# Autodesk Inventor assembly: Assembly1
(part 5 of 8)
- Mate:747: FRAME:1 ↔ disk holder:133
- Mate:748: FRAME:1 ↔ disk holder:134
- Mate:749: FRAME:1 ↔ disk holder:135
- Mate:750: FRAME:1 ↔ disk holder:136
- [RevoluteJoint]: disk holder:137 ↔ coin:137
- [Angle] (-25 deg): disk holder:137 ↔ coin:137
- [Mate]: disk holder:137 ↔ Coil:273
- [Mate]: disk holder:137 ↔ Coil:273
- [Angle] (270 deg): disk holder:137 ↔ Coil:273
- [Mate]: disk holder:137 ↔ Coil:274
- [Angle] (270 deg): disk holder:137 ↔ Coil:274
- [Mate]: disk holder:137 ↔ Coil:274
- [RevoluteJoint]: disk holder:138 ↔ coin:138
- [Angle] (-25 deg): disk holder:138 ↔ coin:138
- [Mate]: disk holder:138 ↔ Coil:275
- [Mate]: disk holder:138 ↔ Coil:275
- [Angle] (270 deg): disk holder:138 ↔ Coil:275
- [Mate]: disk holder:138 ↔ Coil:276
- [Angle] (270 deg): disk holder:138 ↔ Coil:276
- [Mate]: disk holder:138 ↔ Coil:276
- [RevoluteJoint]: disk holder:139 ↔ coin:139
- [Angle] (-25 deg): disk holder:139 ↔ coin:139
- [Mate]: disk holder:139 ↔ Coil:277
- [Mate]: disk holder:139 ↔ Coil:277
- [Angle] (270 deg): disk holder:139 ↔ Coil:277
- [Mate]: disk holder:139 ↔ Coil:278
- [Angle] (270 deg): disk holder:139 ↔ Coil:278
- [Mate]: disk holder:139 ↔ Coil:278
- [RevoluteJoint]: disk holder:140 ↔ coin:140
- [Angle] (-25 deg): disk holder:140 ↔ coin:140
- [Mate]: disk holder:140 ↔ Coil:279
- [Mate]: disk holder:140 ↔ Coil:279
- [Angle] (270 deg): disk holder:140 ↔ Coil:279
- [Mate]: disk holder:140 ↔ Coil:280
- [Angle] (270 deg): disk holder:140 ↔ Coil:280
- [Mate]: disk holder:140 ↔ Coil:280
- [RevoluteJoint]: disk holder:141 ↔ coin:141
- [Angle] (-25 deg): disk holder:141 ↔ coin:141
- [Mate]: disk holder:141 ↔ Coil:281
- [Mate]: disk holder:141 ↔ Coil:281
- [Angle] (270 deg): disk holder:141 ↔ Coil:281
- [Mate]: disk holder:141 ↔ Coil:282
- [Angle] (270 deg): disk holder:141 ↔ Coil:282
- [Mate]: disk holder:141 ↔ Coil:282
- [RevoluteJoint]: disk holder:142 ↔ coin:142
- [Angle] (-25 deg): disk holder:142 ↔ coin:142
- [Mate]: disk holder:142 ↔ Coil:283
- [Mate]: disk holder:142 ↔ Coil:283
- [Angle] (270 deg): disk holder:142 ↔ Coil:283
- [Mate]: disk holder:142 ↔ Coil:284
- [Angle] (270 deg): disk holder:142 ↔ Coil:284
- [Mate]: disk holder:142 ↔ Coil:284
- Flush:213: disk holder:137 ↔ disk holder:138
- Flush:214: disk holder:138 ↔ disk holder:139
- Flush:215: disk holder:139 ↔ disk holder:140
- Flush:216: disk holder:140 ↔ disk holder:141
- Flush:217: disk holder:141 ↔ disk holder:142
- Flush:218: FRAME:1 ↔ disk holder:137
- Flush:219: disk holder:137 ↔ disk holder:138
- Flush:220: disk holder:138 ↔ disk holder:139
- Flush:221: disk holder:139 ↔ disk holder:140
- Flush:222: disk holder:140 ↔ disk holder:141
- Flush:223: disk holder:141 ↔ disk holder:142
- Mate:775: FRAME:1 ↔ disk holder:137
- Mate:776: FRAME:1 ↔ disk holder:137
- Mate:777: FRAME:1 ↔ disk holder:138
- Mate:778: FRAME:1 ↔ disk holder:139
- Mate:779: FRAME:1 ↔ disk holder:140
- Mate:780: FRAME:1 ↔ disk holder:141
- Mate:781: FRAME:1 ↔ disk holder:142
- [RevoluteJoint]: disk holder:143 ↔ coin:143
- [Angle] (-25 deg): disk holder:143 ↔ coin:143
- [Mate]: disk holder:143 ↔ Coil:285
- [Mate]: disk holder:143 ↔ Coil:285
- [Angle] (270 deg): disk holder:143 ↔ Coil:285
- [Mate]: disk holder:143 ↔ Coil:286
- [Angle] (270 deg): disk holder:143 ↔ Coil:286
- [Mate]: disk holder:143 ↔ Coil:286
- [RevoluteJoint]: disk holder:144 ↔ coin:144
- [Angle] (-25 deg): disk holder:144 ↔ coin:144
- [Mate]: disk holder:144 ↔ Coil:287
- [Mate]: disk holder:144 ↔ Coil:287
- [Angle] (270 deg): disk holder:144 ↔ Coil:287
- [Mate]: disk holder:144 ↔ Coil:288
- [Angle] (270 deg): disk holder:144 ↔ Coil:288
- [Mate]: disk holder:144 ↔ Coil:288
- [RevoluteJoint]: disk holder:145 ↔ coin:145
- [Angle] (-25 deg): disk holder:145 ↔ coin:145
- [Mate]: disk holder:145 ↔ Coil:289
- [Mate]: disk holder:145 ↔ Coil:289
- [Angle] (270 deg): disk holder:145 ↔ Coil:289
- [Mate]: disk holder:145 ↔ Coil:290
- [Angle] (270 deg): disk holder:145 ↔ Coil:290
- [Mate]: disk holder:145 ↔ Coil:290
- [RevoluteJoint]: disk holder:146 ↔ coin:146
- [Angle] (-25 deg): disk holder:146 ↔ coin:146
- [Mate]: disk holder:146 ↔ Coil:291
- [Mate]: disk holder:146 ↔ Coil:291
- [Angle] (270 deg): disk holder:146 ↔ Coil:291
- [Mate]: disk holder:146 ↔ Coil:292
- [Angle] (270 deg): disk holder:146 ↔ Coil:292
- [Mate]: disk holder:146 ↔ Coil:292
- [RevoluteJoint]: disk holder:147 ↔ coin:147
- [Angle] (-25 deg): disk holder:147 ↔ coin:147
- [Mate]: disk holder:147 ↔ Coil:293
- [Mate]: disk holder:147 ↔ Coil:293
- [Angle] (270 deg): disk holder:147 ↔ Coil:293
- [Mate]: disk holder:147 ↔ Coil:294
- [Angle] (270 deg): disk holder:147 ↔ Coil:294
- [Mate]: disk holder:147 ↔ Coil:294
- [RevoluteJoint]: disk holder:148 ↔ coin:148
- [Angle] (-25 deg): disk holder:148 ↔ coin:148
- [Mate]: disk holder:148 ↔ Coil:295
- [Mate]: disk holder:148 ↔ Coil:295
- [Angle] (270 deg): disk holder:148 ↔ Coil:295
- [Mate]: disk holder:148 ↔ Coil:296
- [Angle] (270 deg): disk holder:148 ↔ Coil:296
- [Mate]: disk holder:148 ↔ Coil:296
- Flush:224: disk holder:143 ↔ disk holder:144
- Flush:225: disk holder:144 ↔ disk holder:145
- Flush:226: disk holder:145 ↔ disk holder:146
- Flush:227: disk holder:146 ↔ disk holder:147
- Flush:228: disk holder:147 ↔ disk holder:148
- Flush:229: FRAME:1 ↔ disk holder:143
- Mate:806: FRAME:1 ↔ disk holder:143
- Mate:807: disk holder:143 ↔ disk holder:144
- Mate:808: disk holder:144 ↔ disk holder:145
- Mate:809: disk holder:145 ↔ disk holder:146
- Mate:810: disk holder:146 ↔ disk holder:147
- Mate:811: disk holder:147 ↔ disk holder:148
- Mate:812: FRAME:1 ↔ disk holder:143
- Mate:813: FRAME:1 ↔ disk holder:144
- Mate:814: FRAME:1 ↔ disk holder:145
- Mate:815: FRAME:1 ↔ disk holder:146
- Mate:816: FRAME:1 ↔ disk holder:147
- Mate:817: FRAME:1 ↔ disk holder:148
- [RevoluteJoint]: disk holder:149 ↔ coin:149
- [Angle] (-25 deg): disk holder:149 ↔ coin:149
- [Mate]: disk holder:149 ↔ Coil:297
- [Mate]: disk holder:149 ↔ Coil:297
- [Angle] (270 deg): disk holder:149 ↔ Coil:297
- [Mate]: disk holder:149 ↔ Coil:298
- [Angle] (270 deg): disk holder:149 ↔ Coil:298
- [Mate]: disk holder:149 ↔ Coil:298
- [RevoluteJoint]: disk holder:150 ↔ coin:150
- [Angle] (-25 deg): disk holder:150 ↔ coin:150
- [Mate]: disk holder:150 ↔ Coil:299
- [Mate]: disk holder:150 ↔ Coil:299
- [Angle] (270 deg): disk holder:150 ↔ Coil:299
- [Mate]: disk holder:150 ↔ Coil:300
- [Angle] (270 deg): disk holder:150 ↔ Coil:300
- [Mate]: disk holder:150 ↔ Coil:300
- [RevoluteJoint]: disk holder:151 ↔ coin:151
- [Angle] (-25 deg): disk holder:151 ↔ coin:151
- [Mate]: disk holder:151 ↔ Coil:301
- [Mate]: disk holder:151 ↔ Coil:301
- [Angle] (270 deg): disk holder:151 ↔ Coil:301
- [Mate]: disk holder:151 ↔ Coil:302
- [Angle] (270 deg): disk holder:151 ↔ Coil:302
- [Mate]: disk holder:151 ↔ Coil:302
- [RevoluteJoint]: disk holder:152 ↔ coin:152
- [Angle] (-25 deg): disk holder:152 ↔ coin:152
- [Mate]: disk holder:152 ↔ Coil:303
- [Mate]: disk holder:152 ↔ Coil:303
- [Angle] (270 deg): disk holder:152 ↔ Coil:303
- [Mate]: disk holder:152 ↔ Coil:304
- [Angle] (270 deg): disk holder:152 ↔ Coil:304
- [Mate]: disk holder:152 ↔ Coil:304
- [RevoluteJoint]: disk holder:153 ↔ coin:153
- [Angle] (-25 deg): disk holder:153 ↔ coin:153
- [Mate]: disk holder:153 ↔ Coil:305
- [Mate]: disk holder:153 ↔ Coil:305
- [Angle] (270 deg): disk holder:153 ↔ Coil:305
- [Mate]: disk holder:153 ↔ Coil:306
- [Angle] (270 deg): disk holder:153 ↔ Coil:306
- [Mate]: disk holder:153 ↔ Coil:306
- Flush:230: disk holder:149 ↔ disk holder:150
- Flush:231: disk holder:150 ↔ disk holder:151
- Flush:232: disk holder:151 ↔ disk holder:152
- Flush:233: disk holder:152 ↔ disk holder:153
- Flush:234: FRAME:1 ↔ disk holder:149
- Flush:235: disk holder:149 ↔ disk holder:150
- Flush:236: disk holder:150 ↔ disk holder:151
- Flush:237: disk holder:151 ↔ disk holder:152
- Flush:238: disk holder:152 ↔ disk holder:153
- Mate:838: FRAME:1 ↔ disk holder:149
- Mate:839: FRAME:1 ↔ disk holder:149
- Mate:840: FRAME:1 ↔ disk holder:150
- Mate:841: FRAME:1 ↔ disk holder:151
- Mate:842: FRAME:1 ↔ disk holder:152
- Mate:843: FRAME:1 ↔ disk holder:153
- [RevoluteJoint]: disk holder:154 ↔ coin:154
- [Angle] (-25 deg): disk holder:154 ↔ coin:154
- [Mate]: disk holder:154 ↔ Coil:307
- [Mate]: disk holder:154 ↔ Coil:307
- [Angle] (270 deg): disk holder:154 ↔ Coil:307
- [Mate]: disk holder:154 ↔ Coil:308
- [Angle] (270 deg): disk holder:154 ↔ Coil:308
- [Mate]: disk holder:154 ↔ Coil:308
- [RevoluteJoint]: disk holder:155 ↔ coin:155
- [Angle] (-25 deg): disk holder:155 ↔ coin:155
- [Mate]: disk holder:155 ↔ Coil:309
- [Mate]: disk holder:155 ↔ Coil:309
- [Angle] (270 deg): disk holder:155 ↔ Coil:309
- [Mate]: disk holder:155 ↔ Coil:310
- [Angle] (270 deg): disk holder:155 ↔ Coil:310
- [Mate]: disk holder:155 ↔ Coil:310
- [RevoluteJoint]: disk holder:156 ↔ coin:156
- [Angle] (-25 deg): disk holder:156 ↔ coin:156
- [Mate]: disk holder:156 ↔ Coil:311
- [Mate]: disk holder:156 ↔ Coil:311
- [Angle] (270 deg): disk holder:156 ↔ Coil:311
- [Mate]: disk holder:156 ↔ Coil:312
- [Angle] (270 deg): disk holder:156 ↔ Coil:312
- [Mate]: disk holder:156 ↔ Coil:312
- [RevoluteJoint]: disk holder:157 ↔ coin:157
- [Angle] (-25 deg): disk holder:157 ↔ coin:157
- [Mate]: disk holder:157 ↔ Coil:313
- [Mate]: disk holder:157 ↔ Coil:313
- [Angle] (270 deg): disk holder:157 ↔ Coil:313
- [Mate]: disk holder:157 ↔ Coil:314
- [Angle] (270 deg): disk holder:157 ↔ Coil:314
- [Mate]: disk holder:157 ↔ Coil:314
- [RevoluteJoint]: disk holder:158 ↔ coin:158
- [Angle] (-25 deg): disk holder:158 ↔ coin:158
- [Mate]: disk holder:158 ↔ Coil:315
- [Mate]: disk holder:158 ↔ Coil:315
- [Angle] (270 deg): disk holder:158 ↔ Coil:315
- [Mate]: disk holder:158 ↔ Coil:316
- [Angle] (270 deg): disk holder:158 ↔ Coil:316
- [Mate]: disk holder:158 ↔ Coil:316
- Flush:239: disk holder:154 ↔ disk holder:155
- Flush:240: disk holder:155 ↔ disk holder:156
- Flush:241: disk holder:156 ↔ disk holder:157
- Flush:242: disk holder:157 ↔ disk holder:158
- Flush:243: FRAME:1 ↔ disk holder:158
- Flush:244: disk holder:154 ↔ disk holder:155
- Flush:245: disk holder:155 ↔ disk holder:156
- Flush:246: disk holder:156 ↔ disk holder:157
- Flush:247: disk holder:157 ↔ disk holder:158
- Mate:864: FRAME:1 ↔ disk holder:154
- Mate:865: FRAME:1 ↔ disk holder:157
- Mate:866: FRAME:1 ↔ disk holder:157
- Mate:867: FRAME:1 ↔ disk holder:155
- Mate:868: FRAME:1 ↔ disk holder:156
- Mate:869: FRAME:1 ↔ disk holder:158
- [RevoluteJoint]: disk holder:159 ↔ coin:159
- [Angle] (-25 deg): disk holder:159 ↔ coin:159
- [Mate]: disk holder:159 ↔ Coil:317
- [Mate]: disk holder:159 ↔ Coil:317
- [Angle] (270 deg): disk holder:159 ↔ Coil:317
- [Mate]: disk holder:159 ↔ Coil:318
- [Angle] (270 deg): disk holder:159 ↔ Coil:318
- [Mate]: disk holder:159 ↔ Coil:318
- [RevoluteJoint]: disk holder:160 ↔ coin:160
- [Angle] (-25 deg): disk holder:160 ↔ coin:160
- [Mate]: disk holder:160 ↔ Coil:319
- [Mate]: disk holder:160 ↔ Coil:319
- [Angle] (270 deg): disk holder:160 ↔ Coil:319
- [Mate]: disk holder:160 ↔ Coil:320
- [Angle] (270 deg): disk holder:160 ↔ Coil:320
- [Mate]: disk holder:160 ↔ Coil:320
- [RevoluteJoint]: disk holder:161 ↔ coin:161
- [Angle] (-25 deg): disk holder:161 ↔ coin:161
- [Mate]: disk holder:161 ↔ Coil:321
- [Mate]: disk holder:161 ↔ Coil:321
- [Angle] (270 deg): disk holder:161 ↔ Coil:321
- [Mate]: disk holder:161 ↔ Coil:322
- [Angle] (270 deg): disk holder:161 ↔ Coil:322
- [Mate]: disk holder:161 ↔ Coil:322
- [RevoluteJoint]: disk holder:162 ↔ coin:162
- [Angle] (-25 deg): disk holder:162 ↔ coin:162
- [Mate]: disk holder:162 ↔ Coil:323
- [Mate]: disk holder:162 ↔ Coil:323
- [Angle] (270 deg): disk holder:162 ↔ Coil:323
- [Mate]: disk holder:162 ↔ Coil:324
- [Angle] (270 deg): disk holder:162 ↔ Coil:324
- [Mate]: disk holder:162 ↔ Coil:324
- Flush:248: disk holder:159 ↔ disk holder:160
- Flush:249: disk holder:159 ↔ disk holder:161
- Flush:250: disk holder:161 ↔ disk holder:162
- Flush:251: disk holder:159 ↔ disk holder:160
- Flush:252: disk holder:159 ↔ disk holder:161
- Flush:253: disk holder:161 ↔ disk holder:162
- Mate:886: FRAME:1 ↔ disk holder:160
- Mate:887: FRAME:1 ↔ disk holder:160
- Flush:254: FRAME:1 ↔ disk holder:160
- Mate:888: FRAME:1 ↔ disk holder:159
- Mate:889: FRAME:1 ↔ disk holder:161
- Mate:890: FRAME:1 ↔ disk holder:162
- [RevoluteJoint]: disk holder:163 ↔ coin:163
- [Angle] (-25 deg): disk holder:163 ↔ coin:163
- [Mate]: disk holder:163 ↔ Coil:325
- [Mate]: disk holder:163 ↔ Coil:325
- [Angle] (270 deg): disk holder:163 ↔ Coil:325
- [Mate]: disk holder:163 ↔ Coil:326
- [Angle] (270 deg): disk holder:163 ↔ Coil:326
- [Mate]: disk holder:163 ↔ Coil:326
- [RevoluteJoint]: disk holder:164 ↔ coin:164
- [Angle] (-25 deg): disk holder:164 ↔ coin:164
- [Mate]: disk holder:164 ↔ Coil:327
- [Mate]: disk holder:164 ↔ Coil:327
- [Angle] (270 deg): disk holder:164 ↔ Coil:327
- [Mate]: disk holder:164 ↔ Coil:328
- [Angle] (270 deg): disk holder:164 ↔ Coil:328
- [Mate]: disk holder:164 ↔ Coil:328
- [RevoluteJoint]: disk holder:165 ↔ coin:165
- [Angle] (-25 deg): disk holder:165 ↔ coin:165
- [Mate]: disk holder:165 ↔ Coil:329
- [Mate]: disk holder:165 ↔ Coil:329
- [Angle] (270 deg): disk holder:165 ↔ Coil:329
- [Mate]: disk holder:165 ↔ Coil:330
- [Angle] (270 deg): disk holder:165 ↔ Coil:330
- [Mate]: disk holder:165 ↔ Coil:330
- [RevoluteJoint]: disk holder:166 ↔ coin:166
- [Angle] (-25 deg): disk holder:166 ↔ coin:166
- [Mate]: disk holder:166 ↔ Coil:331
- [Mate]: disk holder:166 ↔ Coil:331
- [Angle] (270 deg): disk holder:166 ↔ Coil:331
- [Mate]: disk holder:166 ↔ Coil:332
- [Angle] (270 deg): disk holder:166 ↔ Coil:332
- [Mate]: disk holder:166 ↔ Coil:332
- [RevoluteJoint]: disk holder:167 ↔ coin:167
- [Angle] (-25 deg): disk holder:167 ↔ coin:167
- [Mate]: disk holder:167 ↔ Coil:333
- [Mate]: disk holder:167 ↔ Coil:333
- [Angle] (270 deg): disk holder:167 ↔ Coil:333
- [Mate]: disk holder:167 ↔ Coil:334
- [Angle] (270 deg): disk holder:167 ↔ Coil:334
- [Mate]: disk holder:167 ↔ Coil:334
- [RevoluteJoint]: disk holder:168 ↔ coin:168
- [Angle] (-25 deg): disk holder:168 ↔ coin:168
- [Mate]: disk holder:168 ↔ Coil:335
- [Mate]: disk holder:168 ↔ Coil:335
- [Angle] (270 deg): disk holder:168 ↔ Coil:335
- [Mate]: disk holder:168 ↔ Coil:336
- [Angle] (270 deg): disk holder:168 ↔ Coil:336
- [Mate]: disk holder:168 ↔ Coil:336
- [RevoluteJoint]: disk holder:169 ↔ coin:169
- [Angle] (-25 deg): disk holder:169 ↔ coin:169
- [Mate]: disk holder:169 ↔ Coil:337
- [Mate]: disk holder:169 ↔ Coil:337
- [Angle] (270 deg): disk holder:169 ↔ Coil:337
- [Mate]: disk holder:169 ↔ Coil:338
- [Angle] (270 deg): disk holder:169 ↔ Coil:338
- [Mate]: disk holder:169 ↔ Coil:338
- Flush:255: disk holder:168 ↔ disk holder:169
- Flush:256: disk holder:168 ↔ disk holder:169
- Flush:257: disk holder:163 ↔ disk holder:168
- Flush:258: disk holder:163 ↔ disk holder:167
- Flush:259: disk holder:163 ↔ disk holder:164
- Flush:260: FRAME:1 ↔ disk holder:168
- Flush:261: disk holder:165 ↔ disk holder:167
- Flush:262: disk holder:166 ↔ disk holder:167
- Flush:263: disk holder:163 ↔ disk holder:167
- Flush:264: disk holder:163 ↔ disk holder:166
- Mate:919: FRAME:1 ↔ disk holder:169
- Mate:920: FRAME:1 ↔ disk holder:169
- Mate:921: FRAME:1 ↔ disk holder:168
- Mate:922: FRAME:1 ↔ disk holder:167
- Mate:923: FRAME:1 ↔ disk holder:163
- Mate:924: FRAME:1 ↔ disk holder:163
- Mate:925: FRAME:1 ↔ disk holder:166
- Mate:926: FRAME:1 ↔ disk holder:164
- Mate:927: FRAME:1 ↔ disk holder:164
- Mate:928: FRAME:1 ↔ disk holder:165
- Mate:929: FRAME:1 ↔ disk holder:165
- [RevoluteJoint]: disk holder:170 ↔ coin:170
- [Angle] (-25 deg): disk holder:170 ↔ coin:170
- [Mate]: disk holder:170 ↔ Coil:339
- [Mate]: disk holder:170 ↔ Coil:339
- [Angle] (270 deg): disk holder:170 ↔ Coil:339
- [Mate]: disk holder:170 ↔ Coil:340
- [Angle] (270 deg): disk holder:170 ↔ Coil:340
- [Mate]: disk holder:170 ↔ Coil:340
- [RevoluteJoint]: disk holder:171 ↔ coin:171
- [Angle] (-25 deg): disk holder:171 ↔ coin:171
- [Mate]: disk holder:171 ↔ Coil:341
- [Mate]: disk holder:171 ↔ Coil:341
- [Angle] (270 deg): disk holder:171 ↔ Coil:341
- [Mate]: disk holder:171 ↔ Coil:342
- [Angle] (270 deg): disk holder:171 ↔ Coil:342
- [Mate]: disk holder:171 ↔ Coil:342
- [RevoluteJoint]: disk holder:172 ↔ coin:172
- [Angle] (-25 deg): disk holder:172 ↔ coin:172
- [Mate]: disk holder:172 ↔ Coil:343
- [Mate]: disk holder:172 ↔ Coil:343
- [Angle] (270 deg): disk holder:172 ↔ Coil:343
- [Mate]: disk holder:172 ↔ Coil:344
- [Angle] (270 deg): disk holder:172 ↔ Coil:344
- [Mate]: disk holder:172 ↔ Coil:344
- [RevoluteJoint]: disk holder:173 ↔ coin:173
- [Angle] (-25 deg): disk holder:173 ↔ coin:173
- [Mate]: disk holder:173 ↔ Coil:345
- [Mate]: disk holder:173 ↔ Coil:345
- [Angle] (270 deg): disk holder:173 ↔ Coil:345
- [Mate]: disk holder:173 ↔ Coil:346
- [Angle] (270 deg): disk holder:173 ↔ Coil:346
- [Mate]: disk holder:173 ↔ Coil:346
- [RevoluteJoint]: disk holder:174 ↔ coin:174
- [Angle] (-25 deg): disk holder:174 ↔ coin:174
- [Mate]: disk holder:174 ↔ Coil:347
- [Mate]: disk holder:174 ↔ Coil:347
- [Angle] (270 deg): disk holder:174 ↔ Coil:347
- [Mate]: disk holder:174 ↔ Coil:348
- [Angle] (270 deg): disk holder:174 ↔ Coil:348
- [Mate]: disk holder:174 ↔ Coil:348
- [RevoluteJoint]: disk holder:175 ↔ coin:175
- [Angle] (-25 deg): disk holder:175 ↔ coin:175
- [Mate]: disk holder:175 ↔ Coil:349
- [Mate]: disk holder:175 ↔ Coil:349
- [Angle] (270 deg): disk holder:175 ↔ Coil:349
- [Mate]: disk holder:175 ↔ Coil:350
- [Angle] (270 deg): disk holder:175 ↔ Coil:350
- [Mate]: disk holder:175 ↔ Coil:350
- [RevoluteJoint]: disk holder:176 ↔ coin:176
- [Angle] (-25 deg): disk holder:176 ↔ coin:176
- [Mate]: disk holder:176 ↔ Coil:351
- [Mate]: disk holder:176 ↔ Coil:351
- [Angle] (270 deg): disk holder:176 ↔ Coil:351
- [Mate]: disk holder:176 ↔ Coil:352
- [Angle] (270 deg): disk holder:176 ↔ Coil:352
- [Mate]: disk holder:176 ↔ Coil:352
- [RevoluteJoint]: disk holder:177 ↔ coin:177
- [Angle] (-25 deg): disk holder:177 ↔ coin:177
- [Mate]: disk holder:177 ↔ Coil:353
- [Mate]: disk holder:177 ↔ Coil:353
- [Angle] (270 deg): disk holder:177 ↔ Coil:353
- [Mate]: disk holder:177 ↔ Coil:354
- [Angle] (270 deg): disk holder:177 ↔ Coil:354
- [Mate]: disk holder:177 ↔ Coil:354
- [RevoluteJoint]: disk holder:178 ↔ coin:178
- [Angle] (-25 deg): disk holder:178 ↔ coin:178
- [Mate]: disk holder:178 ↔ Coil:355
- [Mate]: disk holder:178 ↔ Coil:355
- [Angle] (270 deg): disk holder:178 ↔ Coil:355
- [Mate]: disk holder:178 ↔ Coil:356
- [Angle] (270 deg): disk holder:178 ↔ Coil:356
- [Mate]: disk holder:178 ↔ Coil:356
- Flush:265: FRAME:1 ↔ disk holder:172
- Mate:966: FRAME:1 ↔ disk holder:172
- Mate:967: FRAME:1 ↔ disk holder:172
- Flush:266: FRAME:1 ↔ disk holder:171
- Flush:267: disk holder:170 ↔ disk holder:171
- Flush:268: disk holder:170 ↔ disk holder:173
- Flush:269: disk holder:173 ↔ disk holder:174
- Flush:270: disk holder:174 ↔ disk holder:175
- Flush:271: disk holder:175 ↔ disk holder:176
- Flush:272: disk holder:176 ↔ disk holder:177
- Flush:273: disk holder:177 ↔ disk holder:178
- Mate:968: FRAME:1 ↔ disk holder:171
- Mate:969: FRAME:1 ↔ disk holder:171
- Mate:970: FRAME:1 ↔ disk holder:170
- Mate:971: FRAME:1 ↔ disk holder:170
- Mate:972: FRAME:1 ↔ disk holder:173
- Mate:973: FRAME:1 ↔ disk holder:173
- Mate:974: FRAME:1 ↔ disk holder:174
- Mate:975: FRAME:1 ↔ disk holder:174
- Mate:976: FRAME:1 ↔ disk holder:175
- Mate:977: FRAME:1 ↔ disk holder:175
- Mate:978: FRAME:1 ↔ disk holder:176
- Mate:979: FRAME:1 ↔ disk holder:176
- Mate:980: FRAME:1 ↔ disk holder:177
- Mate:981: FRAME:1 ↔ disk holder:177
- Mate:982: FRAME:1 ↔ disk holder:178
- Mate:983: FRAME:1 ↔ disk holder:178
- Mate:984: FRAME:1 ↔ disk holder:42
- Mate:985: FRAME:1 ↔ disk holder:42
- Mate:986: FRAME:1 ↔ disk holder:43
- Mate:987: FRAME:1 ↔ disk holder:43
- Mate:988: FRAME:1 ↔ disk holder:45
- Mate:989: FRAME:1 ↔ disk holder:45